# Autodesk Inventor assembly: Infill3DExtruder
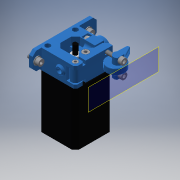
[picture p0: Inventor's stored thumbnail of the model, 180x180]
Saved by Autodesk Inventor 2016 (Build 200138000, 138)
## iProperties
Created: 2015-04-27
Part Number: Infill3DExtruder
Document SubType Name: Assembly
Designer: Jack
Author: Jack
## Documents named in this file (14)
- C:\Users\Jack\ownCloud\Projects\CrossBot\InventorModel\Extruder\Infill3DExtruder\Infill3DExtruderRight.iam
- C:\Users\Jack\ownCloud\Projects\CrossBot\InventorModel\Extruder\Infill3DExtruder\Infill3DBodyRight.ipt
- C:\Users\Jack\ownCloud\Projects\CrossBot\InventorModel\Electronics\Motors\StepperMotorNema17x60mm.ipt
- C:\Users\Jack\ownCloud\Projects\CrossBot\InventorModel\Hardware\Extruder\DriveGearMK8.ipt
- C:\Users\Jack\ownCloud\Projects\CrossBot\InventorModel\Extruder\Infill3DExtruder\Infill3DIdlerRight.ipt
- C:\Users\Jack\ownCloud\Projects\CrossBot\InventorModel\Hardware\Bearing\BearingRadialBall\BearingRadialBall624zz.ipt
- C:\Users\Jack\ownCloud\Projects\CrossBot\InventorModel\Hardware\Nuts\Nut4.ipt
- C:\Users\Jack\ownCloud\Projects\CrossBot\InventorModel\Hardware\BoltWashers\BoltWasher4\BoltWasher4x10.iam
- C:\Users\Jack\ownCloud\Projects\CrossBot\InventorModel\Hardware\Bolts\SHCS\SHCS3\SHCS3x10.ipt
- C:\Users\Jack\ownCloud\Projects\CrossBot\InventorModel\Hardware\Bolts\SHCS\SHCS3\SHCS3x20.ipt
- C:\Users\Jack\ownCloud\Projects\CrossBot\InventorModel\Hardware\Bolts\SHCS\SHCS4\SHCS4x14.ipt
- C:\Users\Jack\ownCloud\Projects\CrossBot\InventorModel\Extruder\Infill3DExtruder\Infill3DExtruderTensionCam.ipt
- C:\Users\Jack\ownCloud\Projects\CrossBot\InventorModel\Extruder\Infill3DExtruder\Infill3DExtruderTensionDowel.ipt
- C:\Users\Jack\ownCloud\Projects\CrossBot\InventorModel\Hardware\Bolts\SHCS\SHCS4\SHCS4x40.ipt
## Components (18 placed, 13 different names)
1. Infill3DBodyRight:1 — Mate:1, Mate:2, Mate:6, Mate:7, Mate:8, Mate:18, Mate:20, Mate:21, Mate:22, Mate:23, Mate:24, Mate:25, Mate:26, Mate:27, Mate:28, Mate:29, Mate:30, Angle:5, Angle:6, Mate:49, Mate:50, Flush:4
2. StepperMotorNema17x60mm:1 — Mate:1, Mate:2, Mate:4, Mate:5, Mate:6
3. DriveGearMK8:1 — Mate:4, Mate:5
4. Infill3DIdlerRight:1 — Mate:7, Mate:8, Mate:9, Mate:10, Mate:11, Angle:4, Mate:37, Mate:38, Mate:39, Tangent:1
5. BearingRadialBall624zz:1 — Mate:9, Mate:10
6. Nut4:1 — Mate:11, Angle:4, Mate:37
7. Nut4:2 — Mate:18, Angle:6, Flush:3
8. Nut4:3 — Mate:20, Angle:5
9. BoltWasher4x10:1 [sub-assembly] — Mate:21, Mate:24
10. BoltWasher4x10:2 [sub-assembly] — Mate:22, Mate:23
11. SHCS3x10:2 — Mate:26, Mate:28
12. SHCS3x10:3 — Mate:25, Mate:27
13. SHCS3x20:1 — Mate:29, Mate:30
14. SHCS4x14:1 — Mate:38, Mate:39
15. Infill3DExtruderTensionCam:1 — Mate:44, Tangent:1, Flush:5
16. Infill3DExtruderTensionDowel:1 — Mate:44, Mate:45, Mate:46, Mate:47, Mate:48, Flush:5
17. SHCS4x40:1 — Mate:45, Mate:47, Mate:49, Flush:3
18. SHCS4x40:2 — Mate:46, Mate:48, Mate:50
## Relationships (39: Mate 32, Angle 3, Flush 3, Tangent 1)
- Mate:1: Infill3DBodyRight:1 ↔ StepperMotorNema17x60mm:1
- Mate:2: Infill3DBodyRight:1 ↔ StepperMotorNema17x60mm:1
- Mate:4: StepperMotorNema17x60mm:1 ↔ DriveGearMK8:1
- Mate:5 (1 mm): StepperMotorNema17x60mm:1 ↔ DriveGearMK8:1
- Mate:6: Infill3DBodyRight:1 ↔ StepperMotorNema17x60mm:1
- Mate:7: Infill3DBodyRight:1 ↔ Infill3DIdlerRight:1
- Mate:8 (0.2 mm): Infill3DBodyRight:1 ↔ Infill3DIdlerRight:1
- Mate:9: Infill3DIdlerRight:1 ↔ BearingRadialBall624zz:1
- Mate:10: Infill3DIdlerRight:1 ↔ BearingRadialBall624zz:1
- Mate:11: Infill3DIdlerRight:1 ↔ Nut4:1
- Mate:18: Infill3DBodyRight:1 ↔ Nut4:2
- Mate:20: Infill3DBodyRight:1 ↔ Nut4:3
- Mate:21: Infill3DBodyRight:1 ↔ BoltWasher4x10:1
- Mate:22: Infill3DBodyRight:1 ↔ BoltWasher4x10:2
- Mate:23: Infill3DBodyRight:1 ↔ BoltWasher4x10:2
- Mate:24: Infill3DBodyRight:1 ↔ BoltWasher4x10:1
- Mate:25: Infill3DBodyRight:1 ↔ SHCS3x10:3
- Mate:26: Infill3DBodyRight:1 ↔ SHCS3x10:2
- Mate:27: Infill3DBodyRight:1 ↔ SHCS3x10:3
- Mate:28: Infill3DBodyRight:1 ↔ SHCS3x10:2
- Mate:29: Infill3DBodyRight:1 ↔ SHCS3x20:1
- Mate:30: Infill3DBodyRight:1 ↔ SHCS3x20:1
- Angle:4 (0 deg): Infill3DIdlerRight:1 ↔ Nut4:1
- Mate:37: Infill3DIdlerRight:1 ↔ Nut4:1
- Mate:38: Infill3DIdlerRight:1 ↔ SHCS4x14:1
- Mate:39: Infill3DIdlerRight:1 ↔ SHCS4x14:1
- Angle:5 (0 deg): Infill3DBodyRight:1 ↔ Nut4:3
- Angle:6 (0 deg): Infill3DBodyRight:1 ↔ Nut4:2
- Mate:44: Infill3DExtruderTensionCam:1 ↔ Infill3DExtruderTensionDowel:1
- Tangent:1: Infill3DIdlerRight:1 ↔ Infill3DExtruderTensionCam:1
- Mate:45: Infill3DExtruderTensionDowel:1 ↔ SHCS4x40:1
- Mate:46: Infill3DExtruderTensionDowel:1 ↔ SHCS4x40:2
- Mate:47: Infill3DExtruderTensionDowel:1 ↔ SHCS4x40:1
- Mate:48: Infill3DExtruderTensionDowel:1 ↔ SHCS4x40:2
- Mate:49: Infill3DBodyRight:1 ↔ SHCS4x40:1
- Mate:50: Infill3DBodyRight:1 ↔ SHCS4x40:2
- Flush:3 (-1 mm): Nut4:2 ↔ SHCS4x40:1
- Flush:4 (-70 mm): Infill3DBodyRight:1
- Flush:5 (7 mm): Infill3DExtruderTensionCam:1 ↔ Infill3DExtruderTensionDowel:1
